# Autodesk Inventor assembly: Assembly_Cube_RaspiCam_v3
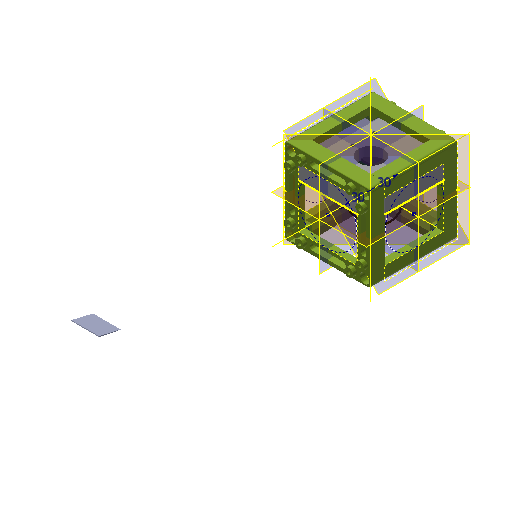
[picture p0: Inventor's stored thumbnail of the model, 512x512]
Saved by Autodesk Inventor 2022 (Build 260153000, 153)
## iProperties
Created: 2019-07-23
Part Number: Assembly_Cube_RaspiCam_v3
Document SubType Name: Assembly
Designer: marsikovabarbora
Mass: 41.4978 g
Surface Area: 307.795 cm^2
Volume: 37.4817 cm^3
Density: 1.10715 g/cm^3
Author: marsikovabarbora
## Documents named in this file (4)
- C:\Users\PrakashLab\Documents\UC2-INVENTOR-Git\uc2_v3\Assembly_Cube_RaspiCam_v3.iam
- C:\Users\PrakashLab\Documents\UC2-INVENTOR-Git\uc2_v3\Assembly_Cube_empty_IM_v3.iam
- C:\Users\PrakashLab\Documents\UC2-INVENTOR-Git\uc2_v3\00_RasPi_Camera.ipt
- C:\Users\PrakashLab\Documents\UC2-INVENTOR-Git\uc2_v3\20_Cube_Insert_RaspiCam_v3.ipt
## Components (3 placed, 3 different names)
1. Assembly_Cube_empty_IM_v3:1 [sub-assembly] — Mate:1, Mate:2, Mate:5, Mate:9, Flush:1, Flush:2
2. 00_RasPi_Camera:1 — Mate:7, Mate:8
3. 20_Cube_Insert_RaspiCam_v3:1 — Mate:7, Mate:8, Mate:9, Flush:1, Flush:2
## Relationships (8: Mate 6, Flush 2)
- Mate:1: Assembly_Cube_empty_IM_v3:1
- Mate:2: Assembly_Cube_empty_IM_v3:1
- Mate:5: Assembly_Cube_empty_IM_v3:1
- Mate:7: 00_RasPi_Camera:1 ↔ 20_Cube_Insert_RaspiCam_v3:1
- Mate:8: 00_RasPi_Camera:1 ↔ 20_Cube_Insert_RaspiCam_v3:1
- Mate:9: Assembly_Cube_empty_IM_v3:1 ↔ 20_Cube_Insert_RaspiCam_v3:1
- Flush:1: Assembly_Cube_empty_IM_v3:1 ↔ 20_Cube_Insert_RaspiCam_v3:1
- Flush:2: Assembly_Cube_empty_IM_v3:1 ↔ 20_Cube_Insert_RaspiCam_v3:1
